# Autodesk Inventor assembly: Assembly1
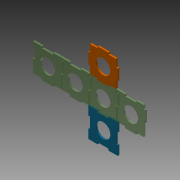
[picture p0: Inventor's stored thumbnail of the model, 180x180]
Saved by Autodesk Inventor 2014 (Build 180170000, 170)
## iProperties
Created: 2014-11-21
Part Number: Assembly1
Document SubType Name: Assembly
Designer: JLM
Author: JLM
## Documents named in this file (4)
- C:\Users\JLM\Documents\Puzzle Box\Assembly1.iam
- C:\Users\JLM\Documents\Puzzle Box\SideA.ipt
- C:\Users\JLM\Documents\Puzzle Box\Top.ipt
- C:\Users\JLM\Documents\Puzzle Box\Bottom.ipt
## Components (6 placed, 3 different names)
1. SideA:1 — Mate:5, Flush:4, Flush:5, Mate:6, Flush:6, Flush:8, Flush:9, Flush:11, Flush:12, Mate:7, Mate:8
2. Top:1 — Mate:6, Flush:6
3. Bottom:1 — Mate:5, Flush:4, Flush:5
4. SideA:2 — Flush:7, Flush:8, Flush:10, Flush:11, Mate:8, Mate:9
5. SideA:3 — Flush:7, Flush:10, Mate:9
6. SideA:4 — Flush:9, Flush:12, Mate:7
## Relationships (14: Flush 9, Mate 5)
- Mate:5: SideA:1 ↔ Bottom:1
- Flush:4: SideA:1 ↔ Bottom:1
- Flush:5: SideA:1 ↔ Bottom:1
- Mate:6: SideA:1 ↔ Top:1
- Flush:6: SideA:1 ↔ Top:1
- Flush:7: SideA:2 ↔ SideA:3
- Flush:8: SideA:1 ↔ SideA:2
- Flush:9: SideA:1 ↔ SideA:4
- Flush:10: SideA:2 ↔ SideA:3
- Flush:11: SideA:1 ↔ SideA:2
- Flush:12: SideA:1 ↔ SideA:4
- Mate:7: SideA:1 ↔ SideA:4
- Mate:8: SideA:1 ↔ SideA:2
- Mate:9: SideA:2 ↔ SideA:3
